# Autodesk Inventor assembly: marco
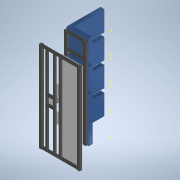
[picture p0: Inventor's stored thumbnail of the model, 180x180]
Saved by Autodesk Inventor 2021.2 (Build 252289000, 289)
## iProperties
Created: 2021-04-11
Part Number: marco
Document SubType Name: Assembly
Designer: equip
Mass: 525959 g
Surface Area: 133006 cm^2
Volume: 315655 cm^3
Density: 1.66625 g/cm^3
_SolveAssemblyDoc: Frame Generator Solve Assembly
_Version: 15.0.0
Author: equip
## Documents named in this file (7)
- C:\Users\equip\Documents\AAA Nacho Mecatrónica\Nacho Sexto Semestre MT\Diseño Mecatrónico\inventor proyecto\marco.iam
- C:\Users\equip\Documents\AAA Nacho Mecatrónica\Nacho Sexto Semestre MT\Diseño Mecatrónico\inventor proyecto\Marco central.ipt
- C:\Users\equip\Documents\AAA Nacho Mecatrónica\Nacho Sexto Semestre MT\Diseño Mecatrónico\inventor proyecto\placa centro.ipt
- C:\Users\equip\Documents\AAA Nacho Mecatrónica\Nacho Sexto Semestre MT\Diseño Mecatrónico\inventor proyecto\Silla del marco.ipt
- C:\Users\equip\Documents\AAA Nacho Mecatrónica\Nacho Sexto Semestre MT\Diseño Mecatrónico\inventor proyecto\marco\Frame\Frame 1619141284633.iam
- C:\Users\equip\Documents\AAA Nacho Mecatrónica\Nacho Sexto Semestre MT\Diseño Mecatrónico\inventor proyecto\placa grande.ipt
- C:\Users\equip\Documents\AAA Nacho Mecatrónica\Nacho Sexto Semestre MT\Diseño Mecatrónico\inventor proyecto\Cilindro\cilindro ensamblaje.iam
## Components (12 placed, 6 different names)
1. Marco central:1
2. placa centro:1 — Coincidencia:10, Coincidencia:11, Nivelación:1, Coincidencia:12
3. Silla del marco:1 — Coincidencia:7, Coincidencia:17, Nivelación:5, Nivelación:6
4. Silla del marco:2 — Coincidencia:7, Coincidencia:8
5. Silla del marco:3 — Coincidencia:8, Coincidencia:9
6. Silla del marco:4 — Coincidencia:9
7. Frame 1619141284633:1 [sub-assembly] — Coincidencia:10, Coincidencia:11, Nivelación:1, Coincidencia:12, Coincidencia:13, Coincidencia:14, Coincidencia:15, Nivelación:2, Coincidencia:16, Nivelación:3, Nivelación:4, Coincidencia:17, Nivelación:5, Nivelación:6, Coincidencia:21, Coincidencia:22, Coincidencia:25, Coincidencia:26
8. placa centro:2 — Coincidencia:13, Coincidencia:14, Coincidencia:15, Nivelación:2, Coincidencia:18, Coincidencia:19, Coincidencia:20
9. placa grande:1 — Coincidencia:16, Nivelación:3, Nivelación:4, Coincidencia:23, Coincidencia:24
10. cilindro ensamblaje:1 [sub-assembly] — Coincidencia:18, Coincidencia:19, Coincidencia:20
11. placa centro:3 — Coincidencia:21, Coincidencia:24, Coincidencia:26
12. placa centro:4 — Coincidencia:22, Coincidencia:23, Coincidencia:25
## Relationships (26: Mate 20, Flush 6)
- Coincidencia:7 [Mate] (105 mm): Silla del marco:1 ↔ Silla del marco:2
- Coincidencia:8 [Mate] (105 mm): Silla del marco:2 ↔ Silla del marco:3
- Coincidencia:9 [Mate] (105 mm): Silla del marco:3 ↔ Silla del marco:4
- Coincidencia:10 [Mate]: placa centro:1 ↔ Frame 1619141284633:1
- Coincidencia:11 [Mate]: placa centro:1 ↔ Frame 1619141284633:1
- Nivelación:1 [Flush] (-2 mm): placa centro:1 ↔ Frame 1619141284633:1
- Coincidencia:12 [Mate] (150 mm): placa centro:1 ↔ Frame 1619141284633:1
- Coincidencia:13 [Mate]: Frame 1619141284633:1 ↔ placa centro:2
- Coincidencia:14 [Mate]: Frame 1619141284633:1 ↔ placa centro:2
- Coincidencia:15 [Mate] (150 mm): Frame 1619141284633:1 ↔ placa centro:2
- Nivelación:2 [Flush] (-2 mm): Frame 1619141284633:1 ↔ placa centro:2
- Coincidencia:16 [Mate]: Frame 1619141284633:1 ↔ placa grande:1
- Nivelación:3 [Flush]: Frame 1619141284633:1 ↔ placa grande:1
- Nivelación:4 [Flush]: Frame 1619141284633:1 ↔ placa grande:1
- Coincidencia:17 [Mate]: Silla del marco:1 ↔ Frame 1619141284633:1
- Nivelación:5 [Flush] (-37.5 mm): Silla del marco:1 ↔ Frame 1619141284633:1
- Nivelación:6 [Flush]: Silla del marco:1 ↔ Frame 1619141284633:1
- Coincidencia:18 [Mate]: placa centro:2 ↔ cilindro ensamblaje:1
- Coincidencia:19 [Mate] (-160 mm): placa centro:2 ↔ cilindro ensamblaje:1
- Coincidencia:20 [Mate] (-122 mm): placa centro:2 ↔ cilindro ensamblaje:1
- Coincidencia:21 [Mate]: Frame 1619141284633:1 ↔ placa centro:3
- Coincidencia:22 [Mate]: Frame 1619141284633:1 ↔ placa centro:4
- Coincidencia:23 [Mate] (25 mm): placa grande:1 ↔ placa centro:4
- Coincidencia:24 [Mate] (25 mm): placa grande:1 ↔ placa centro:3
- Coincidencia:25 [Mate] (40 mm): Frame 1619141284633:1 ↔ placa centro:4
- Coincidencia:26 [Mate] (40 mm): Frame 1619141284633:1 ↔ placa centro:3
## Named parameters: sa_0 = 470880, sa_1 = 470880, sa_2 = 470880, sa_3 = 470880, sa_4 = 1000, sa_5 = 1e+06, sa_6 = 1e+06
note: some values were not read from the file. Shown as the stored number, unit unknown: "sa_0", "sa_1", "sa_2", "sa_3", "sa_4", "sa_5", "sa_6".
